# Autodesk Inventor assembly: ComederoV3
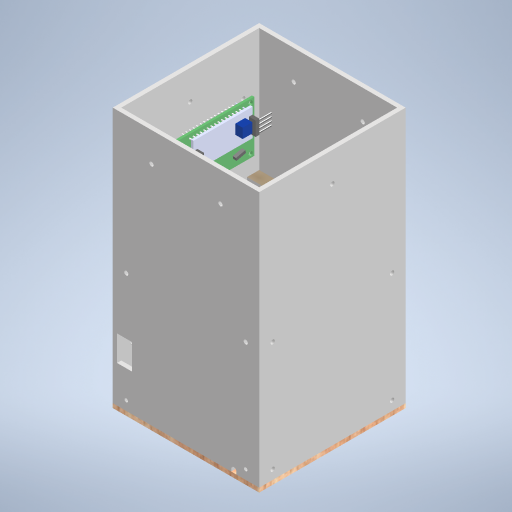
[picture p0: Inventor's stored thumbnail of the model, 512x512]
Saved by Autodesk Inventor 2023 (Build 270158000, 158)
## iProperties
Created: 2022-12-03
Part Number: ComederoV3
Document SubType Name: Assembly
Designer: sergi
Author: sergi
## Documents named in this file (22)
- C:\Users\sergi\OneDrive\Escritorio\Objetos 3d\ComederoV3\ComederoV3.iam
- C:\Users\sergi\OneDrive\Escritorio\Objetos 3d\ComederoV3\Panel1.ipt
- C:\Users\sergi\OneDrive\Escritorio\Objetos 3d\ComederoV3\Panel2.ipt
- C:\Users\sergi\OneDrive\Escritorio\Objetos 3d\ComederoV3\Panel3.ipt
- C:\Users\sergi\OneDrive\Escritorio\Objetos 3d\ComederoV3\Panel4.ipt
- C:\Users\sergi\OneDrive\Escritorio\Objetos 3d\ComederoV3\Escuadra.ipt
- C:\Users\sergi\OneDrive\Escritorio\Objetos 3d\ComederoV3\Escuadra_triple.ipt
- C:\Users\sergi\OneDrive\Escritorio\Objetos 3d\ComederoV3\Embudo.ipt
- C:\Users\sergi\OneDrive\Escritorio\Objetos 3d\ComederoV2\Camisa.ipt
- C:\Users\sergi\OneDrive\Escritorio\Objetos 3d\ComederoV3\Madera intermedia.ipt
- C:\Users\sergi\OneDrive\Escritorio\Objetos 3d\ComederoV3\Tapa_abajo.ipt
- C:\Users\sergi\OneDrive\Escritorio\Cuarto  Carrera\Mecatrónica\Caja conexiones\LCDmodule.ipt
- C:\Users\sergi\OneDrive\Documentos\Inventor\Panel mando.ipt
- C:\Users\sergi\Downloads\Imported Components\Bottom_ULN2003\Bottom_ULN2003.ipt
- C:\Users\sergi\Downloads\Imported Components\Arduino v5\Arduino v5.ipt
- C:\Users\sergi\OneDrive\Escritorio\Objetos 3d\ComederoV3\ComederoV3\Design Accelerator\Engranajes helicoidales3.iam
- C:\Users\sergi\OneDrive\Escritorio\Rodamiento.ipt
- C:\Users\sergi\OneDrive\Escritorio\Objetos 3d\ComederoV3\Soporte mecanismo 2.ipt
- C:\Users\sergi\OneDrive\Escritorio\Objetos 3d\ComederoV3\Soporte mecanismo.ipt
- C:\Users\sergi\OneDrive\Escritorio\Objetos 3d\ComederoV3\MOTOR.ipt
- C:\Users\sergi\OneDrive\Escritorio\Objetos 3d\ComederoV3\Rampa2.ipt
- C:\Users\sergi\OneDrive\Escritorio\Objetos 3d\ComederoV3\Tambor2.ipt
## Components (30 placed, 21 different names)
1. Panel1:1 — Coincidencia:1, Coincidencia:2, Nivelación:1, Nivelación:2, Nivelación:3, Nivelación:4, Nivelación:5, Nivelación:6, Coincidencia:4, Coincidencia:11, Coincidencia:17, Coincidencia:26, Nivelación:19, Nivelación:32
2. Panel2:1 — Coincidencia:1, Coincidencia:3, Nivelación:3, Nivelación:4, Coincidencia:5, Nivelación:7, Coincidencia:8, Nivelación:11, Coincidencia:12, Coincidencia:27, Coincidencia:29, Coincidencia:32, Coincidencia:35, Nivelación:37
3. Panel3:1 — Coincidencia:2, Nivelación:5, Nivelación:6, Coincidencia:6, Nivelación:12, Coincidencia:10, Coincidencia:18, Coincidencia:24
4. Panel4:1 — Coincidencia:3, Nivelación:1, Nivelación:2, Nivelación:8, Coincidencia:7, Coincidencia:9, Coincidencia:23, Coincidencia:30, Nivelación:18, Ángulo:3
5. Escuadra:1 — Coincidencia:16, Coincidencia:17, Coincidencia:18
6. Escuadra_triple:1 — Coincidencia:4, Coincidencia:5, Nivelación:7
7. Escuadra_triple:2 — Nivelación:8, Coincidencia:6, Coincidencia:7
8. Escuadra_triple:3 — Coincidencia:8, Nivelación:11, Coincidencia:9
9. Escuadra_triple:4 — Nivelación:12, Coincidencia:10, Coincidencia:11
10. Embudo:1 — Coincidencia:12, Coincidencia:14
11. Camisa:1 — Coincidencia:14, Nivelación:40
12. Madera intermedia:1 — Coincidencia:16, Coincidencia:22, Coincidencia:25, Coincidencia:28, Coincidencia:44, Coincidencia:54, Coincidencia:59, Nivelación:40, Coincidencia:60, Coincidencia:61, Coincidencia:62
13. Escuadra:2 — Coincidencia:22, Coincidencia:23, Coincidencia:24
14. Escuadra:3 — Coincidencia:25, Coincidencia:26, Coincidencia:27
15. Escuadra:4 — Coincidencia:28, Coincidencia:29, Coincidencia:30
16. Tapa_abajo:1 — Nivelación:18, Nivelación:35
17. LCDmodule:1 — Nivelación:19, Nivelación:32, Coincidencia:32, Coincidencia:33, Nivelación:33, Nivelación:34
18. Panel mando:1 — Coincidencia:33, Nivelación:33, Nivelación:34, Coincidencia:36
19. Bottom_ULN2003:1 — Nivelación:35, Coincidencia:37, Nivelación:36
20. Arduino v5:1 — Coincidencia:35, Coincidencia:36, Coincidencia:37, Nivelación:36, Nivelación:37
21. Rodamiento:1
22. Rodamiento:2 — Coincidencia:47, Coincidencia:48
23. Rodamiento:3 — Coincidencia:44
24. Rodamiento:4
25. Soporte mecanismo 2:1 — Coincidencia:51, Nivelación:39, Coincidencia:56, Ángulo:3
26. Soporte mecanismo:1 — Coincidencia:47, Coincidencia:48, Coincidencia:51, Nivelación:39, Coincidencia:59
27. MOTOR:1 — Coincidencia:56, Coincidencia:58
28. Rampa2:1 — Coincidencia:54, Coincidencia:57, Coincidencia:62
29. Engranajes helicoidales:1 [sub-assembly] — Coincidencia:57, Coincidencia:58
30. Tambor2:1 — Coincidencia:60, Coincidencia:61
## Relationships (63: Mate 42, Flush 20, Angle 1)
- Coincidencia:1 [Mate]: Panel1:1 ↔ Panel2:1
- Coincidencia:2 [Mate]: Panel1:1 ↔ Panel3:1
- Coincidencia:3 [Mate]: Panel2:1 ↔ Panel4:1
- Nivelación:1 [Flush]: Panel1:1 ↔ Panel4:1
- Nivelación:2 [Flush]: Panel1:1 ↔ Panel4:1
- Nivelación:3 [Flush]: Panel1:1 ↔ Panel2:1
- Nivelación:4 [Flush]: Panel1:1 ↔ Panel2:1
- Nivelación:5 [Flush]: Panel1:1 ↔ Panel3:1
- Nivelación:6 [Flush]: Panel1:1 ↔ Panel3:1
- Coincidencia:4 [Mate]: Panel1:1 ↔ Escuadra_triple:1
- Coincidencia:5 [Mate]: Panel2:1 ↔ Escuadra_triple:1
- Nivelación:7 [Flush]: Panel2:1 ↔ Escuadra_triple:1
- Nivelación:8 [Flush]: Panel4:1 ↔ Escuadra_triple:2
- Coincidencia:6 [Mate]: Panel3:1 ↔ Escuadra_triple:2
- Coincidencia:7 [Mate]: Panel4:1 ↔ Escuadra_triple:2
- Coincidencia:8 [Mate]: Panel2:1 ↔ Escuadra_triple:3
- Nivelación:11 [Flush]: Panel2:1 ↔ Escuadra_triple:3
- Coincidencia:9 [Mate]: Panel4:1 ↔ Escuadra_triple:3
- Nivelación:12 [Flush]: Panel3:1 ↔ Escuadra_triple:4
- Coincidencia:10 [Mate]: Panel3:1 ↔ Escuadra_triple:4
- Coincidencia:11 [Mate]: Panel1:1 ↔ Escuadra_triple:4
- Coincidencia:12 [Mate] (-31.5 mm): Panel2:1 ↔ Embudo:1
- Coincidencia:14 [Mate]: Embudo:1 ↔ Camisa:1
- Coincidencia:16 [Mate]: Escuadra:1 ↔ Madera intermedia:1
- Coincidencia:17 [Mate]: Panel1:1 ↔ Escuadra:1
- Coincidencia:18 [Mate]: Panel3:1 ↔ Escuadra:1
- Coincidencia:22 [Mate]: Madera intermedia:1 ↔ Escuadra:2
- Coincidencia:23 [Mate]: Panel4:1 ↔ Escuadra:2
- Coincidencia:24 [Mate]: Panel3:1 ↔ Escuadra:2
- Coincidencia:25 [Mate]: Madera intermedia:1 ↔ Escuadra:3
- Coincidencia:26 [Mate]: Panel1:1 ↔ Escuadra:3
- Coincidencia:27 [Mate]: Panel2:1 ↔ Escuadra:3
- Coincidencia:28 [Mate]: Madera intermedia:1 ↔ Escuadra:4
- Coincidencia:29 [Mate]: Panel2:1 ↔ Escuadra:4
- Coincidencia:30 [Mate]: Panel4:1 ↔ Escuadra:4
- Nivelación:18 [Flush]: Panel4:1 ↔ Tapa_abajo:1
- Nivelación:19 [Flush]: Panel1:1 ↔ LCDmodule:1
- Nivelación:32 [Flush] (35 mm): Panel1:1 ↔ LCDmodule:1
- Coincidencia:32 [Mate] (12.85 mm): Panel2:1 ↔ LCDmodule:1
- Coincidencia:33 [Mate] (35 mm): LCDmodule:1 ↔ Panel mando:1
- Nivelación:33 [Flush]: LCDmodule:1 ↔ Panel mando:1
- Nivelación:34 [Flush]: LCDmodule:1 ↔ Panel mando:1
- Coincidencia:35 [Mate] (5 mm): Panel2:1 ↔ Arduino v5:1
- Coincidencia:36 [Mate] (10 mm): Panel mando:1 ↔ Arduino v5:1
- Nivelación:35 [Flush] (3 mm): Tapa_abajo:1 ↔ Bottom_ULN2003:1
- Coincidencia:37 [Mate] (5 mm): Bottom_ULN2003:1 ↔ Arduino v5:1
- Nivelación:36 [Flush] (-8 mm): Bottom_ULN2003:1 ↔ Arduino v5:1
- Nivelación:37 [Flush] (8 mm): Panel2:1 ↔ Arduino v5:1
- Coincidencia:44 [Mate]: Madera intermedia:1 ↔ Rodamiento:3
- Coincidencia:47 [Mate]: Rodamiento:2 ↔ Soporte mecanismo:1
- Coincidencia:48 [Mate]: Rodamiento:2 ↔ Soporte mecanismo:1
- Coincidencia:51 [Mate]: Soporte mecanismo 2:1 ↔ Soporte mecanismo:1
- Nivelación:39 [Flush]: Soporte mecanismo 2:1 ↔ Soporte mecanismo:1
- Coincidencia:56 [Mate]: Soporte mecanismo 2:1 ↔ MOTOR:1
- Ángulo:3 [Angle] (-90 deg): Panel4:1 ↔ Soporte mecanismo 2:1
- Coincidencia:54 [Mate]: Madera intermedia:1 ↔ Rampa2:1
- Coincidencia:57 [Mate]: Rampa2:1 ↔ Engranajes helicoidales:1
- Coincidencia:58 [Mate]: MOTOR:1 ↔ Engranajes helicoidales:1
- Coincidencia:59 [Mate]: Madera intermedia:1 ↔ Soporte mecanismo:1
- Nivelación:40 [Flush]: Camisa:1 ↔ Madera intermedia:1
- Coincidencia:60 [Mate]: Madera intermedia:1 ↔ Tambor2:1
- Coincidencia:61 [Mate]: Madera intermedia:1 ↔ Tambor2:1
- Coincidencia:62 [Mate]: Madera intermedia:1 ↔ Rampa2:1
